# Autodesk Inventor assembly: SCSW12-8
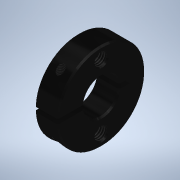
[picture p0: Inventor's stored thumbnail of the model, 180x180]
Saved by Autodesk Inventor 2022 (Build 260153000, 153)
## iProperties
Part Number: SCSW12-8
Catalog Web Link: www.cadenas.de
Description: SCSW, PSCSW, SSCSW, SCSWA, SCSWAW-Set Collars - Slit 2 Hole/2 Tap - Standard Type - 2 Tap Type
Vendor: MISUMI
Document SubType Name: Assembly
Designer: partserver
Manufacturer: MISUMI
Mass: 4.23513 g
Surface Area: 28.6495 cm^2
Volume: 4.23513 cm^3
Density: 1 g/cm^3
Category: PARTsolutions
Company: MISUMI
PSOL_IDENT_0: {$CADENAS_DATA\23d-libs\misumi\metric\03_set_collars\scsw_asmtab.prj},208 {VTYP=3D},{STYP=ASSTAB},{N
PSOL_IDENT_1: B=SCSW12-8},{LINA=SCSW12-8},{NN=SCSW, PSCSW, SSCSW, SCSWA, SCSWAW},{DATE=30.11.2021 05:42:05},{GEOMD
PSOL_IDENT_2: ATE=15.09.2021 06:02:54},{VERSION=},{LINEID=70},{WBVAR=MAT,ST,BS},{WBNUMERIC=BS}  {NB=SCSW12-8},{LIN
PSOL_IDENT_3: A=SCSW12-8},{KT=DUMMY},{PN=SCSW12-8},{TYPE=SCSW},{MAT=1045},{MATA='1045','S45C Equivalent','304','SU
PSOL_IDENT_4: S304 Equivalent','2017','2017 Aluminum Alloy'},{ST=Black Oxide},{AC=Hexagon Socket Head Set Screw 1
PSOL_IDENT_5: Pc.},{D=12},{BS=8},{B1=8,10,12,15},{D1=30},{M=M3},{THMD=3},{THDMIN=2.459},{ST0='Black Oxide','Black
PSOL_IDENT_6: Oxide','Electroless Nickel Plating','Electroless Nickel Plating'},{DD=3.4},{R=3.00},{W=1.5},{X=10.0}
PSOL_IDENT_7: ,{Y=5.0},{Z=9~10},{S=5.5},{P=22},{C=0.5},{L=12},{M1=M5},{ZZ=9.5},{THMD1=5},{THDMIN1=4.134},{PPATH=sc
PSOL_IDENT_8: sw_templ.prj}
NB: SCSW12-8
NN: SCSW, PSCSW, SSCSW, SCSWA, SCSWAW
NT: Set Collars - Slit 2 Hole/2 Tap - Standard Type - 2 Tap Type
NBSYN: $PN.
LINA: SCSW12-8
CATALOG: Misumi
PN: SCSW12-8
MAT: S45C Equivalent
ST: Black Oxide
AC: Hexagon Socket Head Set Screw 1 Pc.
D: 12
BS: 8
D1: 30
M: M3
DD: 3.4
R: 3
W: 1.5
X: 10
Y: 5
Z: 9~10
S: 5.5
P: 22
M1: M5
SUPPLIER: MISUMI
ARTICLENO: SCSW12-8
BOMINFO: SCSW12-8
CREATOR: CADENAS GmbH
Title: SCSW12-8
Author: Cadenas PARTsolutions
Comments: Set Collars - Slit 2 Hole/2 Tap - Standard Type - 2 Tap Type
## Documents named in this file (3)
- C:\Users\rkawaba1\Documents\GrabCAD\NHK2022\BasicParts\SetCollar\SCSW12-8\SCSW12-8.iam
- C:\Users\rkawaba1\Documents\GrabCAD\NHK2022\BasicParts\SetCollar\SCSW12-8\SCSW12-8b.ipt
- C:\Users\rkawaba1\Documents\GrabCAD\NHK2022\BasicParts\SetCollar\SCSW12-8\Slotted head cap screw ISO 4762 - M3x12.ipt
## Components (2 placed, 2 different names)
1. SCSW12-8b:1 — body_screw_Z@1 <-> IP1_Z@2
2. Slotted head cap screw ISO 4762 - M3x12:1 — body_screw_Z@1 <-> IP1_Z@2
## Relationships (1: Mate 1)
- body_screw_Z@1 <-> IP1_Z@2 [Mate]: SCSW12-8b:1 ↔ Slotted head cap screw ISO 4762 - M3x12:1
